# Autodesk Inventor assembly: circularholder_assembly
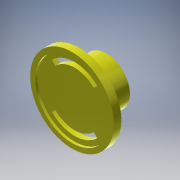
[picture p0: Inventor's stored thumbnail of the model, 180x180]
Saved by Autodesk Inventor 2019 (Build 230136000, 136)
## iProperties
Created: 2019-02-20
Part Number: circularholder_assembly
Document SubType Name: Assembly
Designer: jmc
Author: jmc
## Documents named in this file (4)
- C:\Users\l0086\Desktop\Models\Stamp\circularholder_assembly.iam
- C:\Users\l0086\Desktop\Models\Stamp\circularholder.ipt
- C:\Users\l0086\Desktop\Models\Stamp\nut_adapter.ipt
- C:\Users\l0086\Desktop\Models\Stamp\Part2.ipt
## Components (3 placed, 3 different names)
1. circularholder:1 — Rigid:1
2. nut_adapter:1 — Rigid:1
3. Part2:1
## Relationships (1: WeldJoint 1)
- Rigid:1 [WeldJoint]: circularholder:1 ↔ nut_adapter:1
